# Autodesk Inventor assembly: CL2-100
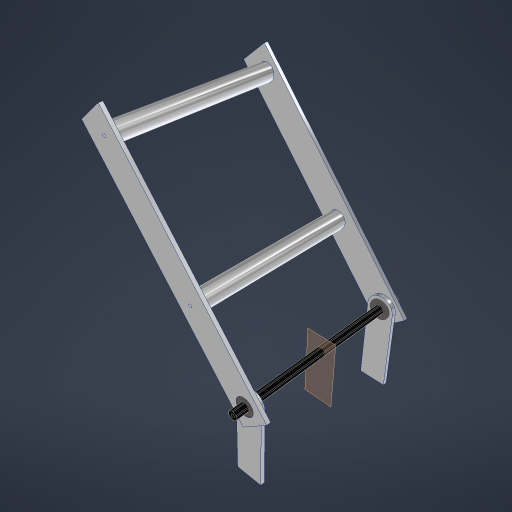
[picture p0: Inventor's stored thumbnail of the model, 512x512]
Saved by Autodesk Inventor 2023.4 (Build 274418000, 418)
## iProperties
Created: 2025-01-26
Part Number: CL2-100
Document SubType Name: Assembly
Designer: brand
Author: brand
## Documents named in this file (6)
- C:\Users\brand\OneDrive\Documents\GitHub\robotics 23\2025-ReefScape---CAD\Climber\CL2\CL2-100.iam
- C:\Users\brand\OneDrive\Documents\GitHub\robotics 23\2025-ReefScape---CAD\Climber\CL2\CL2-001.ipt
- C:\Users\brand\OneDrive\Documents\GitHub\robotics 23\2025-ReefScape---CAD\COMMON PARTS\BEARINGS\0_500_Hex_ID_x_1_125_OD_x_0_313_WD_Flanged_Bearing_v2_217-3875.ipt
- C:\Users\brand\OneDrive\Documents\GitHub\robotics 23\2025-ReefScape---CAD\Climber\CL2\CL2-002.ipt
- C:\Users\brand\OneDrive\Documents\GitHub\robotics 23\2025-ReefScape---CAD\Climber\CL2\CL2-003.ipt
- C:\Users\brand\OneDrive\Documents\GitHub\robotics 23\2025-ReefScape---CAD\Climber\CL2\CL2-004.ipt
## Components (11 placed, 5 different names)
1. CL2-001:1 — Mate:2, Symmetry:1
2. CL2-001:2 — Mate:2, Symmetry:1
3. 0_500_Hex_ID_x_1_125_OD_x_0_313_WD_Flanged_Bearing_v2_217-3875:1
4. 0_500_Hex_ID_x_1_125_OD_x_0_313_WD_Flanged_Bearing_v2_217-3875:2 — Mate:3
5. CL2-002:1 — Insert:3, Insert:6, Mate:5
6. CL2-002:2 — Insert:4, Insert:5
7. CL2-003:1 — Mate:3, Flush:1, Mate:4
8. CL2-004:1 — Insert:3, Insert:4, Insert:8
9. CL2-004:2 — Insert:5, Insert:6, Insert:7
10. 0_500_Hex_ID_x_1_125_OD_x_0_313_WD_Flanged_Bearing_v2_217-3875:3 — Insert:8, Mate:4
11. 0_500_Hex_ID_x_1_125_OD_x_0_313_WD_Flanged_Bearing_v2_217-3875:4 — Insert:7
## Relationships (16: Insert 8, Mate 5, Angle 1, Symmetry 1, Flush 1)
- [Mate]: CL2-001:1 ↔ CL2-001:2
- [Angle] (0 deg): CL2-001:1 ↔ CL2-001:2
- [Insert]: CL2-001:2 ↔ 0_500_Hex_ID_x_1_125_OD_x_0_313_WD_Flanged_Bearing_v2_217-3875:1
- [Insert]: CL2-001:1 ↔ 0_500_Hex_ID_x_1_125_OD_x_0_313_WD_Flanged_Bearing_v2_217-3875:2
- Mate:2 (-254 mm): CL2-001:1 ↔ CL2-001:2
- Mate:3: 0_500_Hex_ID_x_1_125_OD_x_0_313_WD_Flanged_Bearing_v2_217-3875:2 ↔ CL2-003:1
- Symmetry:1: CL2-001:1 ↔ CL2-001:2
- Flush:1: CL2-003:1
- Insert:3: CL2-002:1 ↔ CL2-004:1
- Insert:4: CL2-002:2 ↔ CL2-004:1
- Insert:5: CL2-002:2 ↔ CL2-004:2
- Insert:6: CL2-002:1 ↔ CL2-004:2
- Insert:7: CL2-004:2 ↔ 0_500_Hex_ID_x_1_125_OD_x_0_313_WD_Flanged_Bearing_v2_217-3875:4
- Insert:8: CL2-004:1 ↔ 0_500_Hex_ID_x_1_125_OD_x_0_313_WD_Flanged_Bearing_v2_217-3875:3
- Mate:4: CL2-003:1 ↔ 0_500_Hex_ID_x_1_125_OD_x_0_313_WD_Flanged_Bearing_v2_217-3875:3
- Mate:5: CL2-002:1
